# Autodesk Inventor assembly: Manipulator_Sterowniki_Robotow_II_czlon
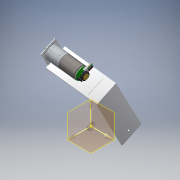
[picture p0: Inventor's stored thumbnail of the model, 180x180]
Saved by Autodesk Inventor 2019 (Build 230136000, 136)
## iProperties
Created: 2021-05-21
Part Number: Manipulator_Sterowniki_Robotow_II_czlon
Document SubType Name: Assembly
Designer: DOMEK
Sending System: SIEMENS PLM Software NX 1907
Preprocessor: ST-DEVELOPER v16.7
Title: Manipulator_Sterowniki_Robotów.stp
## Documents named in this file (4)
- D:\Manipulator\Inventor-20\Manipulator_Sterowniki_Robotow_II_czlon.iam
- D:\Manipulator\Inventor-20\Manipulator_Handler_Silnikow.ipt
- D:\Manipulator\Inventor-20\25d-metal-gearmotor-172-227-encoder.ipt
- D:\Manipulator\Inventor-20\Manipulator_DrugiStopien.ipt
## Components (3 placed, 3 different names)
1. Manipulator_DrugiStopien:1 — Mate:1, Flush:1, Flush:5
2. Manipulator_Handler_Silnikow:2 — Mate:1, Flush:1, Insert:7, Insert:8, Flush:5
3. 25d-metal-gearmotor-172-227-encoder:2 — Insert:7, Insert:8
## Relationships (5: Flush 2, Insert 2, Mate 1)
- Mate:1: Manipulator_DrugiStopien:1 ↔ Manipulator_Handler_Silnikow:2
- Flush:1: Manipulator_DrugiStopien:1 ↔ Manipulator_Handler_Silnikow:2
- Insert:7: Manipulator_Handler_Silnikow:2 ↔ 25d-metal-gearmotor-172-227-encoder:2
- Insert:8: Manipulator_Handler_Silnikow:2 ↔ 25d-metal-gearmotor-172-227-encoder:2
- Flush:5 (4 mm): Manipulator_DrugiStopien:1 ↔ Manipulator_Handler_Silnikow:2
